# Autodesk Inventor assembly: LegInnerGear
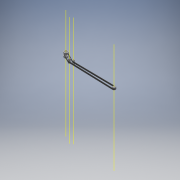
[picture p0: Inventor's stored thumbnail of the model, 180x180]
Saved by Autodesk Inventor 2019.1 (Build 231200000, 200)
## iProperties
Created: 2018-11-28
Part Number: LegInnerGear
Material: Generisch
Document SubType Name: Assembly
Designer: JochenAlt
Author: JochenAlt
## Documents named in this file (3)
- D:\Projects\Ondine\CAD\Leg\LegInnerGear.iam
- D:\Projects\Ondine\CAD\Leg\LegInnerGear\Übertragung des Zahnriemens1.iam
- D:\Projects\Ondine\CAD\Leg\LegInnerGear\InnerGearForm.ipt
## Components (2 placed, 2 different names)
1. Übertragung des Zahnriemens:1 [sub-assembly] — Passend:2, Passend:3
2. InnerGearForm:1 — Fluchtend:1, Passend:2, Passend:3
## Relationships (3: Mate 2, Flush 1)
- Fluchtend:1 [Flush]: InnerGearForm:1
- Passend:2 [Mate]: Übertragung des Zahnriemens:1 ↔ InnerGearForm:1
- Passend:3 [Mate]: Übertragung des Zahnriemens:1 ↔ InnerGearForm:1
